# Autodesk Inventor assembly: main assembly
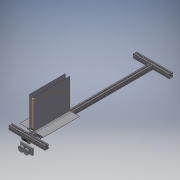
[picture p0: Inventor's stored thumbnail of the model, 180x180]
Saved by Autodesk Inventor 2016 SP1 (Build 200210100, 210)
## iProperties
Created: 2016-05-25
Part Number: main assembly
Document SubType Name: Assembly
Designer: ubik
Author: ubik
## Documents named in this file (18)
- E:\GitHub\glue-filter\hardware\inventor\main assembly.iam
- E:\GitHub\glue-filter\hardware\inventor\Linear Rail.ipt
- E:\GitHub\glue-filter\hardware\inventor\Carriage.ipt
- E:\GitHub\glue-filter\hardware\inventor\30x30\30x30-01.ipt
- E:\GitHub\glue-filter\hardware\inventor\30x30.ipt
- E:\GitHub\glue-filter\hardware\inventor\mobile bottom plate.ipt
- E:\GitHub\glue-filter\hardware\inventor\mobile vertical plate.ipt
- E:\GitHub\glue-filter\hardware\inventor\mobile top plate.ipt
- E:\GitHub\glue-filter\hardware\inventor\filter base.ipt
- E:\GitHub\glue-filter\hardware\inventor\filter top plate.ipt
- E:\GitHub\glue-filter\hardware\inventor\filter top.ipt
- E:\GitHub\glue-filter\hardware\inventor\gear.ipt
- E:\GitHub\glue-filter\hardware\inventor\6000-Bearing.ipt
- E:\GitHub\glue-filter\hardware\inventor\bearing support.ipt
- E:\GitHub\glue-filter\hardware\inventor\sheet support.ipt
- E:\GitHub\glue-filter\hardware\inventor\NEMA17 Stepper.ipt
- E:\GitHub\glue-filter\hardware\inventor\nema17 x plate.ipt
- E:\GitHub\glue-filter\hardware\inventor\30x30\30x30-02.ipt
## Components (22 placed, 16 different names)
1. Linear Rail:1 — Tangent:1, Tangent:2, Angle:1, Angle:2, Mate:1, Mate:2, Mate:4, Flush:3, Flush:4
2. Carriage:1 — Tangent:1, Tangent:2, Angle:1, Angle:2, Flush:1, Flush:2, Mate:1, Mate:2, Mate:3, Mate:5, Flush:5, Flush:6
3. Carriage:2 — Flush:1, Flush:2, Mate:3, Mate:6
4. 30x30-01:1 — Mate:4, Flush:3, Flush:4, Mate:26, Flush:24, Flush:25, Mate:27, Flush:26, Flush:27, Flush:29, Mate:28
5. mobile bottom plate:1 — Mate:5, Flush:5, Mate:6, Flush:6, Mate:7, Flush:7, Flush:8, Mate:8, Flush:9, Flush:10
6. mobile vertical plate:1 — Mate:7, Flush:7, Flush:9, Flush:12, Mate:9
7. mobile vertical plate:2 — Flush:8, Mate:8, Flush:10, Flush:11
8. mobile top plate:1 — Flush:11, Flush:12, Mate:9, Mate:10, Flush:13, Flush:14
9. filter base:1 — Mate:11, Mate:12, Mate:13, Mate:14, Flush:15, Flush:16, Mate:20, Mate:23
10. filter top plate:1 — Mate:10, Flush:13, Flush:14, Mate:11, Mate:12, Mate:13, Flush:21
11. filter top:1 — Mate:14, Flush:15, Flush:16, Mate:21, Mate:22
12. gear:1 — Tangent:3, Flush:17, Mate:15, Mate:19
13. gear:2 — Tangent:3, Flush:17, Mate:16
14. 6000-Bearing:1 — Mate:15, Flush:18, Mate:17, Flush:19, Flush:20, Mate:19
15. 6000-Bearing:2 — Mate:16, Flush:18, Flush:20, Mate:18
16. bearing support:1 — Mate:17, Flush:19, Mate:18
17. sheet support:1 — Mate:20, Mate:21, Flush:22
18. sheet support:2 — Mate:22, Mate:23, Flush:21, Flush:22
19. NEMA17 Stepper:1 — Flush:23, Mate:24, Mate:25
20. nema17 x plate:1 — Flush:23, Mate:24, Mate:25, Mate:26, Flush:24, Flush:25
21. 30x30-02:3 — Mate:27, Flush:26, Flush:28, Flush:29
22. 30x30-02:4 — Flush:27, Flush:28, Mate:28
## Relationships (62: Flush 29, Mate 28, Tangent 3, Angle 2)
- Tangent:1: Linear Rail:1 ↔ Carriage:1
- Tangent:2: Linear Rail:1 ↔ Carriage:1
- Angle:1 (0 deg): Linear Rail:1 ↔ Carriage:1
- Angle:2 (0 deg): Linear Rail:1 ↔ Carriage:1
- Flush:1: Carriage:1 ↔ Carriage:2
- Flush:2: Carriage:1 ↔ Carriage:2
- Mate:1 (0.5 mm): Linear Rail:1 ↔ Carriage:1
- Mate:2 (1 mm): Linear Rail:1 ↔ Carriage:1
- Mate:3 (110 mm): Carriage:1 ↔ Carriage:2
- Mate:4: Linear Rail:1 ↔ 30x30-01:1
- Flush:3 (9 mm): Linear Rail:1 ↔ 30x30-01:1
- Flush:4: Linear Rail:1 ↔ 30x30-01:1
- Mate:5: Carriage:1 ↔ mobile bottom plate:1
- Flush:5 (4 mm): Carriage:1 ↔ mobile bottom plate:1
- Mate:6: Carriage:2 ↔ mobile bottom plate:1
- Flush:6: Carriage:1 ↔ mobile bottom plate:1
- Mate:7: mobile bottom plate:1 ↔ mobile vertical plate:1
- Flush:7: mobile bottom plate:1 ↔ mobile vertical plate:1
- Flush:8: mobile bottom plate:1 ↔ mobile vertical plate:2
- Mate:8: mobile bottom plate:1 ↔ mobile vertical plate:2
- Flush:9: mobile bottom plate:1 ↔ mobile vertical plate:1
- Flush:10: mobile bottom plate:1 ↔ mobile vertical plate:2
- Flush:11: mobile vertical plate:2 ↔ mobile top plate:1
- Flush:12 (-10 mm): mobile vertical plate:1 ↔ mobile top plate:1
- Mate:9: mobile vertical plate:1 ↔ mobile top plate:1
- Mate:10: mobile top plate:1 ↔ filter top plate:1
- Flush:13 (50 mm): mobile top plate:1 ↔ filter top plate:1
- Flush:14 (2 mm): mobile top plate:1 ↔ filter top plate:1
- Mate:11: filter base:1 ↔ filter top plate:1
- Mate:12: filter base:1 ↔ filter top plate:1
- Mate:13: filter base:1 ↔ filter top plate:1
- Mate:14: filter base:1 ↔ filter top:1
- Flush:15 (-11 mm): filter base:1 ↔ filter top:1
- Flush:16 (10 mm): filter base:1 ↔ filter top:1
- Tangent:3: gear:1 ↔ gear:2
- Flush:17: gear:1 ↔ gear:2
- Mate:15 (2 mm): gear:1 ↔ 6000-Bearing:1
- Mate:16: gear:2 ↔ 6000-Bearing:2
- Flush:18: 6000-Bearing:1 ↔ 6000-Bearing:2
- Mate:17: 6000-Bearing:1 ↔ bearing support:1
- Flush:19: 6000-Bearing:1 ↔ bearing support:1
- Flush:20: 6000-Bearing:1 ↔ 6000-Bearing:2
- Mate:18: 6000-Bearing:2 ↔ bearing support:1
- Mate:19: gear:1 ↔ 6000-Bearing:1
- Mate:20: filter base:1 ↔ sheet support:1
- Mate:21: filter top:1 ↔ sheet support:1
- Mate:22: filter top:1 ↔ sheet support:2
- Mate:23: filter base:1 ↔ sheet support:2
- Flush:21: filter top plate:1 ↔ sheet support:2
- Flush:22: sheet support:1 ↔ sheet support:2
- Flush:23: NEMA17 Stepper:1 ↔ nema17 x plate:1
- Mate:24: NEMA17 Stepper:1 ↔ nema17 x plate:1
- Mate:25: NEMA17 Stepper:1 ↔ nema17 x plate:1
- Mate:26: 30x30-01:1 ↔ nema17 x plate:1
- Flush:24: 30x30-01:1 ↔ nema17 x plate:1
- Flush:25: 30x30-01:1 ↔ nema17 x plate:1
- Mate:27: 30x30-01:1 ↔ 30x30-02:3
- Flush:26: 30x30-01:1 ↔ 30x30-02:3
- Flush:27: 30x30-01:1 ↔ 30x30-02:4
- Flush:28: 30x30-02:3 ↔ 30x30-02:4
- Flush:29 (135 mm): 30x30-01:1 ↔ 30x30-02:3
- Mate:28: 30x30-01:1 ↔ 30x30-02:4
